# Autodesk Inventor assembly: Walls
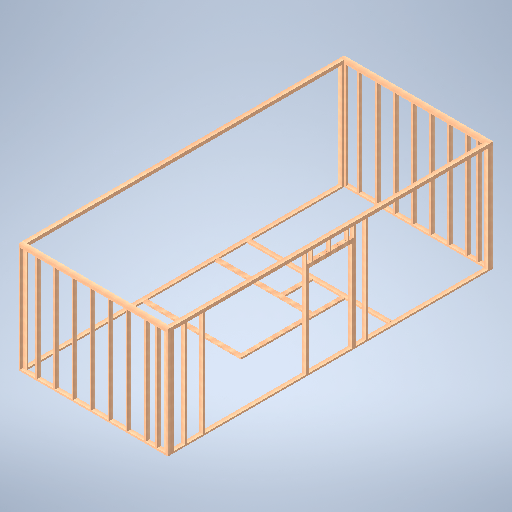
[picture p0: Inventor's stored thumbnail of the model, 512x512]
Saved by Autodesk Inventor 2025.1 (Build 291241020, 241B)
## iProperties
Created: 2024-09-15
Part Number: Walls
Document SubType Name: Assembly
Designer: Tom
Author: Tom
## Documents named in this file (14)
- C:\Users\Tom\Documents\Inventor\Mobility\Additional_Building\Framing_For_First_Floor.iam
- C:\Users\Tom\Documents\Inventor\Mobility\Additional_Building\Plate_With_Length_144_Inches.ipt
- C:\Users\Tom\Documents\Inventor\Mobility\Additional_Building\Plate_With_Length_125_Inches.ipt
- C:\Users\Tom\Documents\Inventor\Mobility\Additional_Building\California_Corner.iam
- C:\Users\Tom\Documents\Inventor\Mobility\Additional_Building\Stud_With_Height_93_Inches.ipt
- C:\Users\Tom\Documents\Inventor\Mobility\Additional_Building\Plate_With_Length_132_Inches.ipt
- C:\Users\Tom\Documents\Inventor\Mobility\Additional_Building\Plate_With_Length_68.5_Inches.ipt
- C:\Users\Tom\Documents\Inventor\Mobility\Additional_Building\Plate_With_Length_86.5625_Inches_And_Image_Of_Bath_Tub.ipt
- C:\Users\Tom\Documents\Inventor\Mobility\Additional_Building\Plate_With_Length_60_Inches.ipt
- C:\Users\Tom\Documents\Inventor\Mobility\Additional_Building\Plate_With_Length_25_Inches.ipt
- C:\Users\Tom\Documents\Inventor\Mobility\Additional_Building\Plate_With_Length_86.5625_Inches.ipt
- C:\Users\Tom\Documents\Inventor\Mobility\Additional_Building\Header_With_Dimensions_3.5_x_3.5_x_41.25_Inches.iam
- C:\Users\Tom\Documents\Inventor\Mobility\Additional_Building\Stud_With_Height_80.5_Inches.ipt
- C:\Users\Tom\Documents\Inventor\Mobility\Additional_Building\Stud_With_Height_9_Inches.ipt
## Components (57 placed, 13 different names)
1. California_Corner:1 [sub-assembly] — Mate:2, Flush:3, Flush:4
2. California_Corner:2 [sub-assembly] — Mate:13, Flush:13, Flush:14, Flush:19, Flush:20, Flush:31, Mate:34
3. California_Corner:3 [sub-assembly] — Mate:14, Flush:15, Flush:16
4. California_Corner:4 [sub-assembly] — Mate:15, Flush:17, Flush:18
5. Plate_With_Length_125_Inches:5 — Mate:16, Flush:22, Mate:17, Mate:19, Mate:24, Flush:27
6. Plate_With_Length_60_Inches:1 — Mate:19, Mate:27, Mate:31
7. Plate_With_Length_25_Inches:1 — Mate:25, Mate:28
8. Plate_With_Length_25_Inches:2 — Mate:24, Flush:27, Mate:25, Mate:29
9. Plate_With_Length_86.5625_Inches_And_Image_Of_Bath_Tub:1 — Mate:26, Flush:28, Mate:27, Mate:28, Mate:29
10. Plate_With_Length_86.5625_Inches:1 — Mate:30, Mate:31, Flush:29
11. Stud_With_Height_93_Inches:56 — Mate:33, Flush:32, Mate:34, Mate:35, Flush:33, Mate:39
12. Header_With_Dimensions_3.5_x_3.5_x_41.25_Inches:1 [sub-assembly] — Mate:35, Flush:33, Flush:34, Mate:37, Mate:42, Flush:38
13. Stud_With_Height_93_Inches:57 — Mate:36, Flush:35, Mate:37, Mate:41
14. Stud_With_Height_80.5_Inches:1 — Mate:38, Flush:36, Mate:39
15. Stud_With_Height_80.5_Inches:2 — Mate:40, Flush:37, Mate:41
16. Stud_With_Height_93_Inches:58 — Mate:44, Flush:42, Flush:43
17. Plate_With_Length_132_Inches:1 — Mate:8, Flush:9, Flush:10, Mate:10
18. Plate_With_Length_132_Inches:2
19. Plate_With_Length_144_Inches:9 — Mate:11, Mate:12, Flush:12
20. Plate_With_Length_144_Inches:10
21. Stud_With_Height_93_Inches:49 — Mate:32, Flush:30, Flush:31
22. Stud_With_Height_93_Inches:50
23. Stud_With_Height_93_Inches:1 — Mate:4, Flush:6, Flush:19, Flush:39, Flush:43
24. Stud_With_Height_93_Inches:51
25. Stud_With_Height_9_Inches:1 — Mate:42, Flush:38, Flush:39
26. Stud_With_Height_9_Inches:2
27. Stud_With_Height_9_Inches:3
28. Plate_With_Length_144_Inches:1 — Flush:5, Mate:15, Flush:17, Flush:18, Mate:30, Flush:29
29. Plate_With_Length_144_Inches:2 — Mate:14, Flush:15, Flush:16, Mate:26, Flush:28
30. Plate_With_Length_144_Inches:3 — Mate:1, Flush:1, Flush:2, Mate:4, Flush:6, Mate:13, Flush:13, Flush:14, Mate:16, Flush:22, Mate:33, Flush:32, Flush:34, Mate:38, Flush:36
31. Plate_With_Length_144_Inches:4 — Mate:2, Flush:3, Flush:4, Mate:36, Flush:35, Mate:40, Flush:37, Mate:44, Flush:42
32. Plate_With_Length_125_Inches:1 — Mate:1, Flush:1, Flush:2, Mate:3, Mate:7, Mate:32, Flush:30
33. Plate_With_Length_125_Inches:2 — Mate:17
34. Plate_With_Length_144_Inches:5 — Flush:9
35. Plate_With_Length_144_Inches:6
36. Plate_With_Length_144_Inches:7 — Mate:9, Flush:11
37. Plate_With_Length_144_Inches:8 — Mate:11, Flush:12
38. Plate_With_Length_125_Inches:3 — Flush:7, Mate:8, Flush:10
39. Plate_With_Length_125_Inches:4
40. Stud_With_Height_93_Inches:23 — Flush:7, Mate:7, Flush:20
41. Stud_With_Height_93_Inches:24
42. Stud_With_Height_93_Inches:25
43. Stud_With_Height_93_Inches:26
44. Stud_With_Height_93_Inches:27
45. Stud_With_Height_93_Inches:45
46. Stud_With_Height_93_Inches:46
47. Stud_With_Height_93_Inches:28
48. Stud_With_Height_93_Inches:29
49. Stud_With_Height_93_Inches:30
50. Stud_With_Height_93_Inches:31
51. Stud_With_Height_93_Inches:32
52. Stud_With_Height_93_Inches:47
53. Stud_With_Height_93_Inches:48
54. Plate_With_Length_68.5_Inches:1 — Mate:9, Mate:10, Flush:11
55. Plate_With_Length_68.5_Inches:2 — Mate:12
56. Plate_With_Length_68.5_Inches:3
57. Plate_With_Length_68.5_Inches:4
## Component patterns: (2 elements), (2 elements), (2 elements, first: Plate_With_Length_132_Inches:1), (2 elements, first: Plate_With_Length_144_Inches:9), (2 elements, first: Stud_With_Height_93_Inches:49), (2 elements, first: Stud_With_Height_93_Inches:1), (3 elements, first: Stud_With_Height_9_Inches:1), (4 elements, first: Plate_With_Length_144_Inches:1), (2 elements, first: Plate_With_Length_125_Inches:1), Component Pattern 1:2 (4 elements), Component Pattern 2:2 (2 elements), (7 elements, first: Stud_With_Height_93_Inches:23), Component Pattern 6:2 (7 elements), (2 elements, first: Plate_With_Length_68.5_Inches:1), Component Pattern 10:2 (2 elements)
## Relationships (71: Mate 36, Flush 35)
- Mate:1: Plate_With_Length_144_Inches:3 ↔ Plate_With_Length_125_Inches:1
- Flush:1: Plate_With_Length_144_Inches:3 ↔ Plate_With_Length_125_Inches:1
- Flush:2: Plate_With_Length_144_Inches:3 ↔ Plate_With_Length_125_Inches:1
- Mate:2: California_Corner:1 ↔ Plate_With_Length_144_Inches:4
- Flush:3: California_Corner:1 ↔ Plate_With_Length_144_Inches:4
- Flush:4: California_Corner:1 ↔ Plate_With_Length_144_Inches:4
- Flush:5: Plate_With_Length_144_Inches:1
- Mate:3 (1536.7 mm): Plate_With_Length_125_Inches:1
- Mate:4: Stud_With_Height_93_Inches:1 ↔ Plate_With_Length_144_Inches:3
- Flush:6: Stud_With_Height_93_Inches:1 ↔ Plate_With_Length_144_Inches:3
- Flush:7: Plate_With_Length_125_Inches:3 ↔ Stud_With_Height_93_Inches:23
- Mate:7: Plate_With_Length_125_Inches:1 ↔ Stud_With_Height_93_Inches:23
- Mate:8: Plate_With_Length_132_Inches:1 ↔ Plate_With_Length_125_Inches:3
- Flush:9: Plate_With_Length_132_Inches:1 ↔ Plate_With_Length_144_Inches:5
- Flush:10: Plate_With_Length_132_Inches:1 ↔ Plate_With_Length_125_Inches:3
- Mate:9: Plate_With_Length_144_Inches:7 ↔ Plate_With_Length_68.5_Inches:1
- Mate:10: Plate_With_Length_132_Inches:1 ↔ Plate_With_Length_68.5_Inches:1
- Flush:11: Plate_With_Length_144_Inches:7 ↔ Plate_With_Length_68.5_Inches:1
- Mate:11: Plate_With_Length_144_Inches:9 ↔ Plate_With_Length_144_Inches:8
- Mate:12: Plate_With_Length_144_Inches:9 ↔ Plate_With_Length_68.5_Inches:2
- Flush:12: Plate_With_Length_144_Inches:9 ↔ Plate_With_Length_144_Inches:8
- Mate:13: California_Corner:2 ↔ Plate_With_Length_144_Inches:3
- Flush:13: California_Corner:2 ↔ Plate_With_Length_144_Inches:3
- Flush:14: California_Corner:2 ↔ Plate_With_Length_144_Inches:3
- Mate:14: California_Corner:3 ↔ Plate_With_Length_144_Inches:2
- Flush:15: California_Corner:3 ↔ Plate_With_Length_144_Inches:2
- Flush:16: California_Corner:3 ↔ Plate_With_Length_144_Inches:2
- Mate:15: California_Corner:4 ↔ Plate_With_Length_144_Inches:1
- Flush:17: California_Corner:4 ↔ Plate_With_Length_144_Inches:1
- Flush:18: California_Corner:4 ↔ Plate_With_Length_144_Inches:1
- Flush:19 (387.35 mm): California_Corner:2 ↔ Stud_With_Height_93_Inches:1
- Flush:20 (501.65 mm): California_Corner:2 ↔ Stud_With_Height_93_Inches:23
- Mate:16: Plate_With_Length_125_Inches:5 ↔ Plate_With_Length_144_Inches:3
- Flush:22: Plate_With_Length_125_Inches:5 ↔ Plate_With_Length_144_Inches:3
- Mate:17 (2092.325 mm): Plate_With_Length_125_Inches:5 ↔ Plate_With_Length_125_Inches:2
- Mate:19 (723.9 mm): Plate_With_Length_125_Inches:5 ↔ Plate_With_Length_60_Inches:1
- Mate:24: Plate_With_Length_125_Inches:5 ↔ Plate_With_Length_25_Inches:2
- Flush:27: Plate_With_Length_125_Inches:5 ↔ Plate_With_Length_25_Inches:2
- Mate:25 (635 mm): Plate_With_Length_25_Inches:1 ↔ Plate_With_Length_25_Inches:2
- Mate:26: Plate_With_Length_86.5625_Inches_And_Image_Of_Bath_Tub:1 ↔ Plate_With_Length_144_Inches:2
- Flush:28: Plate_With_Length_86.5625_Inches_And_Image_Of_Bath_Tub:1 ↔ Plate_With_Length_144_Inches:2
- Mate:27: Plate_With_Length_60_Inches:1 ↔ Plate_With_Length_86.5625_Inches_And_Image_Of_Bath_Tub:1
- Mate:28: Plate_With_Length_25_Inches:1 ↔ Plate_With_Length_86.5625_Inches_And_Image_Of_Bath_Tub:1
- Mate:29: Plate_With_Length_25_Inches:2 ↔ Plate_With_Length_86.5625_Inches_And_Image_Of_Bath_Tub:1
- Mate:30: Plate_With_Length_86.5625_Inches:1 ↔ Plate_With_Length_144_Inches:1
- Mate:31: Plate_With_Length_60_Inches:1 ↔ Plate_With_Length_86.5625_Inches:1
- Flush:29: Plate_With_Length_86.5625_Inches:1 ↔ Plate_With_Length_144_Inches:1
- Mate:32: Stud_With_Height_93_Inches:49 ↔ Plate_With_Length_125_Inches:1
- Flush:30: Stud_With_Height_93_Inches:49 ↔ Plate_With_Length_125_Inches:1
- Flush:31 (250.825 mm): California_Corner:2 ↔ Stud_With_Height_93_Inches:49
- Mate:33: Stud_With_Height_93_Inches:56 ↔ Plate_With_Length_144_Inches:3
- Flush:32: Stud_With_Height_93_Inches:56 ↔ Plate_With_Length_144_Inches:3
- Mate:34 (-3133.725 mm): California_Corner:2 ↔ Stud_With_Height_93_Inches:56
- Mate:35: Stud_With_Height_93_Inches:56 ↔ Header_With_Dimensions_3.5_x_3.5_x_41.25_Inches:1
- Flush:33: Stud_With_Height_93_Inches:56 ↔ Header_With_Dimensions_3.5_x_3.5_x_41.25_Inches:1
- Flush:34 (2082.8 mm): Header_With_Dimensions_3.5_x_3.5_x_41.25_Inches:1 ↔ Plate_With_Length_144_Inches:3
- Mate:36: Stud_With_Height_93_Inches:57 ↔ Plate_With_Length_144_Inches:4
- Flush:35: Stud_With_Height_93_Inches:57 ↔ Plate_With_Length_144_Inches:4
- Mate:37: Header_With_Dimensions_3.5_x_3.5_x_41.25_Inches:1 ↔ Stud_With_Height_93_Inches:57
- Mate:38: Stud_With_Height_80.5_Inches:1 ↔ Plate_With_Length_144_Inches:3
- Flush:36: Stud_With_Height_80.5_Inches:1 ↔ Plate_With_Length_144_Inches:3
- Mate:39: Stud_With_Height_93_Inches:56 ↔ Stud_With_Height_80.5_Inches:1
- Mate:40: Stud_With_Height_80.5_Inches:2 ↔ Plate_With_Length_144_Inches:4
- Flush:37: Stud_With_Height_80.5_Inches:2 ↔ Plate_With_Length_144_Inches:4
- Mate:41: Stud_With_Height_93_Inches:57 ↔ Stud_With_Height_80.5_Inches:2
- Mate:42: Header_With_Dimensions_3.5_x_3.5_x_41.25_Inches:1 ↔ Stud_With_Height_9_Inches:1
- Flush:38: Header_With_Dimensions_3.5_x_3.5_x_41.25_Inches:1 ↔ Stud_With_Height_9_Inches:1
- Flush:39 (2844.8 mm): Stud_With_Height_93_Inches:1 ↔ Stud_With_Height_9_Inches:1
- Mate:44: Stud_With_Height_93_Inches:58 ↔ Plate_With_Length_144_Inches:4
- Flush:42: Stud_With_Height_93_Inches:58 ↔ Plate_With_Length_144_Inches:4
- Flush:43 (4064 mm): Stud_With_Height_93_Inches:58 ↔ Stud_With_Height_93_Inches:1
